# Autodesk Inventor assembly: Glue Reservoir Plate - V2
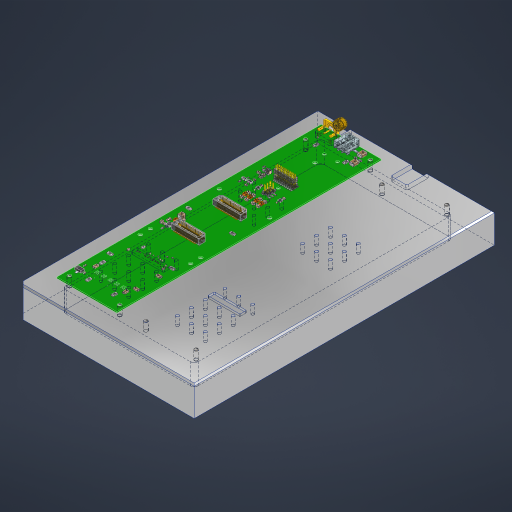
[picture p0: Inventor's stored thumbnail of the model, 512x512]
Saved by Autodesk Inventor 2024 (Build 280153000, 153)
## iProperties
Created: 2022-02-14
Part Number: Glue Reservoir Plate - V2
Document SubType Name: Assembly
Designer: Caleb
Author: Caleb
## Documents named in this file (4)
- C:\Users\cfangmeier3\Desktop\nebraska-silicon-lab\Hardware\ETL\Module Assembly\Module PCB V0 Wirebonding Plate V1\Module PCB V0 Wirebonding Plate V1.iam
- C:\Users\cfangmeier3\Desktop\nebraska-silicon-lab\Hardware\ETL\Module Assembly\Module PCB V0 Wirebonding Plate V1\Module PCB V0 Wirebonding Plate V1.ipt
- C:\Users\cfangmeier3\Desktop\nebraska-silicon-lab\Hardware\ETL\Module Assembly\Module PCB V0 Wirebonding Plate V1\ETROC2_V0\ETROC2_V0.iam
- C:\Users\cfangmeier3\Desktop\nebraska-silicon-lab\Hardware\ETL\Module Assembly\Module PCB V0 Wirebonding Plate V1\91595A103_Dowel Pin\91595A103_Dowel Pin.ipt
## Components (10 placed, 3 different names)
1. Module PCB V0 Wirebonding Plate V1:1 — Mate:1, Angle:1, Insert:5, Insert:6, Insert:7, Insert:8, Insert:9, Insert:10, Insert:11, Insert:12, Insert:13
2. ETROC2_V0:1 [sub-assembly] — Mate:1, Angle:1, Insert:5
3. 91595A103_Dowel Pin:1 — Insert:9
4. 91595A103_Dowel Pin:2 — Insert:6
5. 91595A103_Dowel Pin:3 — Insert:7
6. 91595A103_Dowel Pin:4 — Insert:8
7. 91595A103_Dowel Pin:5 — Insert:10
8. 91595A103_Dowel Pin:6 — Insert:11
9. 91595A103_Dowel Pin:7 — Insert:12
10. 91595A103_Dowel Pin:8 — Insert:13
## Relationships (11: Insert 9, Mate 1, Angle 1)
- Mate:1: Module PCB V0 Wirebonding Plate V1:1 ↔ ETROC2_V0:1
- Angle:1 (0 deg): Module PCB V0 Wirebonding Plate V1:1 ↔ ETROC2_V0:1
- Insert:5: Module PCB V0 Wirebonding Plate V1:1 ↔ ETROC2_V0:1
- Insert:6: Module PCB V0 Wirebonding Plate V1:1 ↔ 91595A103_Dowel Pin:2
- Insert:7 (-0.355 mm): Module PCB V0 Wirebonding Plate V1:1 ↔ 91595A103_Dowel Pin:3
- Insert:8 (-0.355 mm): Module PCB V0 Wirebonding Plate V1:1 ↔ 91595A103_Dowel Pin:4
- Insert:9 (-0.355 mm): Module PCB V0 Wirebonding Plate V1:1 ↔ 91595A103_Dowel Pin:1
- Insert:10 (-0.355 mm): Module PCB V0 Wirebonding Plate V1:1 ↔ 91595A103_Dowel Pin:5
- Insert:11 (-0.355 mm): Module PCB V0 Wirebonding Plate V1:1 ↔ 91595A103_Dowel Pin:6
- Insert:12 (-0.355 mm): Module PCB V0 Wirebonding Plate V1:1 ↔ 91595A103_Dowel Pin:7
- Insert:13 (-0.355 mm): Module PCB V0 Wirebonding Plate V1:1 ↔ 91595A103_Dowel Pin:8
